# Autodesk Inventor assembly: Spool_B
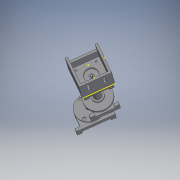
[picture p0: Inventor's stored thumbnail of the model, 180x180]
Saved by Autodesk Inventor 2017 (Build 210142000, 142)
## iProperties
Created: 2017-04-30
Part Number: Spool_B
Document SubType Name: Assembly
Designer: s4321966
Author: s4321966
## Documents named in this file (9)
- \\puffball.labs.eait.uq.edu.au\s4321966\Documents\GitHub\METR4810\Mechanical\metr4810_spool draft\metr4810_spool draft\PARTS\Spool_B.iam
- \\puffball.labs.eait.uq.edu.au\s4321966\Documents\GitHub\METR4810\Mechanical\metr4810_spool draft\metr4810_spool draft\PARTS\Slipring_mount.ipt
- \\puffball.labs.eait.uq.edu.au\s4321966\Documents\GitHub\METR4810\Mechanical\metr4810_spool draft\metr4810_spool draft\PARTS\SlipRing-022A-12.ipt
- \\puffball.labs.eait.uq.edu.au\s4321966\Documents\GitHub\METR4810\Mechanical\metr4810_spool draft\metr4810_spool draft\PARTS\SpoolMount.ipt
- \\puffball.labs.eait.uq.edu.au\s4321966\Documents\GitHub\METR4810\Mechanical\metr4810_spool draft\metr4810_spool draft\std_bearing.ipt
- \\puffball.labs.eait.uq.edu.au\s4321966\Documents\GitHub\METR4810\Mechanical\spool\stepperMount.ipt
- \\puffball.labs.eait.uq.edu.au\s4321966\Documents\GitHub\METR4810\Mechanical\metr4810_spool draft\metr4810_spool draft\PARTS\Spool_revB1.ipt
- \\puffball.labs.eait.uq.edu.au\s4321966\Documents\GitHub\METR4810\Mechanical\metr4810_spool draft\metr4810_spool draft\PARTS\Spool_revB2.ipt
- \\puffball.labs.eait.uq.edu.au\s4321966\Documents\GitHub\METR4810\Mechanical\metr4810_spool draft\metr4810_spool draft\PARTS\Spool_revB3.ipt
## Components (10 placed, 8 different names)
1. SlipRing-022A-12:1 — Mate:6, Tangent:4, Mate:8
2. std_bearing:1 — Insert:5, Tangent:6, Mate:7, Tangent:7
3. std_bearing:2 — Tangent:3, Mate:3, Tangent:5
4. stepperMount:1 — Insert:5, Flush:2, Flush:3
5. Slipring_mount:1 — Mate:6, Tangent:4, Flush:1
6. Spool_revB1:1 — Mate:1, Tangent:1, Tangent:3, Mate:3, Mate:4
7. Spool_revB2:1 — Mate:2, Tangent:2, Mate:5, Mate:7, Tangent:7
8. Spool_revB3:1 — Mate:1, Mate:2, Tangent:1, Tangent:2
9. SpoolMount:1 — Mate:4, Tangent:5, Flush:1, Flush:2, Mate:8
10. SpoolMount:2 — Mate:5, Tangent:6, Flush:3
## Relationships (19: Mate 8, Tangent 7, Flush 3, Insert 1)
- Insert:5: std_bearing:1 ↔ stepperMount:1
- Mate:1: Spool_revB1:1 ↔ Spool_revB3:1
- Mate:2: Spool_revB2:1 ↔ Spool_revB3:1
- Tangent:1: Spool_revB1:1 ↔ Spool_revB3:1
- Tangent:2: Spool_revB2:1 ↔ Spool_revB3:1
- Tangent:3: std_bearing:2 ↔ Spool_revB1:1
- Mate:3: std_bearing:2 ↔ Spool_revB1:1
- Mate:4: Spool_revB1:1 ↔ SpoolMount:1
- Mate:5: Spool_revB2:1 ↔ SpoolMount:2
- Mate:6: SlipRing-022A-12:1 ↔ Slipring_mount:1
- Tangent:4: SlipRing-022A-12:1 ↔ Slipring_mount:1
- Tangent:5: std_bearing:2 ↔ SpoolMount:1
- Tangent:6: std_bearing:1 ↔ SpoolMount:2
- Mate:7: std_bearing:1 ↔ Spool_revB2:1
- Tangent:7: std_bearing:1 ↔ Spool_revB2:1
- Flush:1: Slipring_mount:1 ↔ SpoolMount:1
- Flush:2: stepperMount:1 ↔ SpoolMount:1
- Flush:3: stepperMount:1 ↔ SpoolMount:2
- Mate:8: SlipRing-022A-12:1 ↔ SpoolMount:1
